# Autodesk Inventor assembly: Arem2
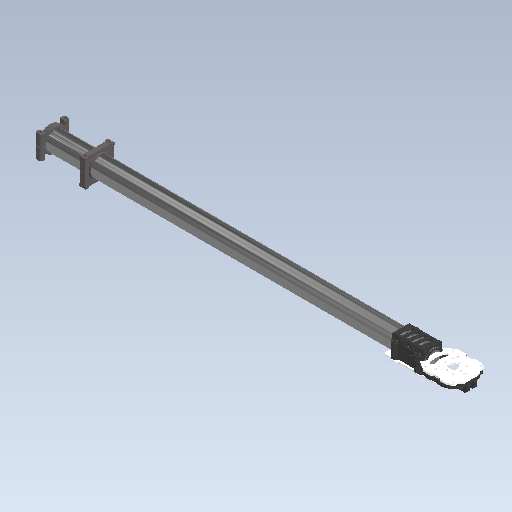
[picture p0: Inventor's stored thumbnail of the model, 512x512]
Saved by Autodesk Inventor 2020.2 (Build 242310000, 310)
## iProperties
Created: 2020-04-17
Part Number: Arem2
Document SubType Name: Assembly
Designer: Muhyidin
Author: Muhyidin
## Documents named in this file (5)
- D:\Google Drive\UVa\Research\PhD Research\Drone-Project\Drone-project-CAD\CAD Files\Tarot 810\Arem2.iam
- D:\Google Drive\UVa\Research\PhD Research\Drone-Project\Drone-project-CAD\CAD Files\Tarot 810\tube.ipt
- D:\Google Drive\UVa\Research\PhD Research\Drone-Project\Drone-project-CAD\CAD Files\Tarot 810\Tarot 25MM Tube Clamp Metal TL80b03.ipt
- D:\Google Drive\UVa\Research\PhD Research\Drone-Project\Drone-project-CAD\CAD Files\Tarot 810\Držák motoru.iam
- D:\Google Drive\UVa\Research\PhD Research\Drone-Project\Drone-project-CAD\CAD Files\Tarot 810\clamp nganu.ipt
## Components (6 placed, 4 different names)
1. tube:1 — Rotational:4, Rotational:5, Rotational:6, Rotational:7, Rotational:8
2. Tarot 25MM Tube Clamp Metal TL80b03:3 — Rotational:5
3. Tarot 25MM Tube Clamp Metal TL80b03:4 — Rotational:4
4. Držák motoru:1 [sub-assembly] — Rotational:6
5. clamp nganu:1 — Rotational:8
6. clamp nganu:2 — Rotational:7
## Relationships (5: RevoluteJoint 5)
- Rotational:4 [RevoluteJoint] (56.5 mm): tube:1 ↔ Tarot 25MM Tube Clamp Metal TL80b03:4
- Rotational:5 [RevoluteJoint] (56.5 mm): tube:1 ↔ Tarot 25MM Tube Clamp Metal TL80b03:3
- Rotational:6 [RevoluteJoint]: tube:1 ↔ Držák motoru:1
- Rotational:7 [RevoluteJoint]: tube:1 ↔ clamp nganu:2
- Rotational:8 [RevoluteJoint]: tube:1 ↔ clamp nganu:1
